# Autodesk Inventor assembly: ABD_Version_0.1_leftleg
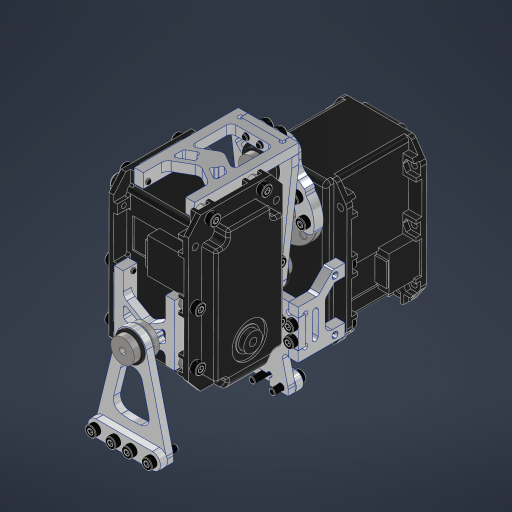
[picture p0: Inventor's stored thumbnail of the model, 512x512]
Saved by Autodesk Inventor 2024 (Build 280153000, 153)
## iProperties
Created: 2024-01-23
Part Number: ABD_Version_0.1_leftleg
Document SubType Name: Assembly
Designer: ASUS
Mass: 357.136 g
Surface Area: 604.848 cm^2
Volume: 181.423 cm^3
Density: 1.96853 g/cm^3
Author: ASUS
## Documents named in this file (10)
- C:\Users\ASUS\Desktop\Anti_Backlash_Structure_OP\v3_Frame\ABD_V3_Left_OP.iam
- C:\Users\ASUS\Desktop\Anti_Backlash_Structure_OP\v3_Frame\Roll_Fixation_Set.iam
- C:\Users\ASUS\Desktop\Anti_Backlash_Structure_OP\v3_Frame\ABD_MX_64_Roll_Fixation_Set.iam
- C:\Users\ASUS\Desktop\Anti_Backlash_Structure_OP\v3_Frame\ABD_MX_64_Slider_Fixation_Set_Right2Horn.iam
- C:\Users\ASUS\Desktop\Anti_Backlash_Structure_OP\v3_Frame\ABD_Slider_Set_v3.iam
- C:\Users\ASUS\Desktop\Anti_Backlash_Structure_OP\MISUMI\C-WSSA12-4-2.ipt
- C:\Users\ASUS\Desktop\Anti_Backlash_Structure_OP\MISUMI\NBW-0612-10.ipt
- C:\Users\ASUS\Desktop\Anti_Backlash_Structure_OP\MISUMI\LED-0606.ipt
- C:\Users\ASUS\Desktop\Anti_Backlash_Structure_OP\v3_Frame\Ubber_Washer_1.5mm.ipt
- C:\Users\ASUS\Desktop\Anti_Backlash_Structure_OP\MISUMI\DBB4-8-5.ipt
## Components (10 placed, 9 different names)
1. Roll_Fixation_Set:1 [sub-assembly] — 삽입:5, 메이트:13
2. ABD_MX_64_Roll_Fixation_Set:1 [sub-assembly] — 메이트:2, 삽입:5, 메이트:10, 메이트:11
3. ABD_MX_64_Slider_Fixation_Set_Right2Horn:1 [sub-assembly] — 메이트:2, 메이트:4, 메이트:5, 메이트:10, 메이트:11
4. LED-0606:1 — 삽입:9, 메이트:5, 삽입:15
5. Ubber_Washer_1.5mm:1 — 삽입:9, 메이트:4, 삽입:10
6. DBB4-8-5:1 — 삽입:11, 메이트:12
7. NBW-0612-10:1 — 삽입:13, 삽입:15
8. C-WSSA12-4-2:1 — 삽입:13, 삽입:16
9. NBW-0612-10:2 — 삽입:10, 삽입:11
10. ABD_Slider_Set_v3:1 [sub-assembly] — 메이트:12, 삽입:16, 메이트:13
## Relationships (14: Mate 7, Insert 7)
- 메이트:2 [Mate] (0.05 mm): ABD_MX_64_Roll_Fixation_Set:1 ↔ ABD_MX_64_Slider_Fixation_Set_Right2Horn:1
- 삽입:5 [Insert]: Roll_Fixation_Set:1 ↔ ABD_MX_64_Roll_Fixation_Set:1
- 삽입:9 [Insert]: LED-0606:1 ↔ Ubber_Washer_1.5mm:1
- 메이트:4 [Mate]: ABD_MX_64_Slider_Fixation_Set_Right2Horn:1 ↔ Ubber_Washer_1.5mm:1
- 메이트:5 [Mate] (0.025 mm): ABD_MX_64_Slider_Fixation_Set_Right2Horn:1 ↔ LED-0606:1
- 삽입:10 [Insert]: Ubber_Washer_1.5mm:1 ↔ NBW-0612-10:2
- 삽입:11 [Insert]: DBB4-8-5:1 ↔ NBW-0612-10:2
- 삽입:13 [Insert]: NBW-0612-10:1 ↔ C-WSSA12-4-2:1
- 메이트:10 [Mate]: ABD_MX_64_Roll_Fixation_Set:1 ↔ ABD_MX_64_Slider_Fixation_Set_Right2Horn:1
- 메이트:11 [Mate]: ABD_MX_64_Roll_Fixation_Set:1 ↔ ABD_MX_64_Slider_Fixation_Set_Right2Horn:1
- 메이트:12 [Mate]: DBB4-8-5:1 ↔ ABD_Slider_Set_v3:1
- 삽입:15 [Insert]: LED-0606:1 ↔ NBW-0612-10:1
- 삽입:16 [Insert]: C-WSSA12-4-2:1 ↔ ABD_Slider_Set_v3:1
- 메이트:13 [Mate]: Roll_Fixation_Set:1 ↔ ABD_Slider_Set_v3:1
